# Autodesk Inventor assembly: project_maket
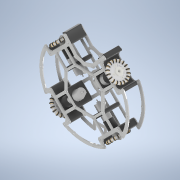
[picture p0: Inventor's stored thumbnail of the model, 180x180]
Saved by Autodesk Inventor 2020 (Build 240168000, 168)
## iProperties
Created: 2024-02-27
Part Number: project_maket
Document SubType Name: Assembly
Designer: 4s
Author: 4s
## Documents named in this file (9)
- C:\Users\4s\Documents\Inventor models\Asterisk\robot_v2\project_maket.iam
- C:\Users\4s\Documents\Inventor models\Asterisk\robot_v2\bottom_plate.ipt
- C:\Users\4s\Documents\Inventor models\Asterisk\robot_v2\motor mounts\mid_mount.ipt
- C:\Users\4s\Documents\Inventor models\Asterisk\robot_v2\motor mounts\left_motor_v2.ipt
- C:\Users\4s\Documents\Inventor models\Asterisk\robot_v2\motor mounts\right_motor_v2.ipt
- C:\Users\4s\Documents\Inventor models\Asterisk\robot_v2\motor mounts\back_motor_short.ipt
- C:\Users\4s\Documents\Inventor models\Asterisk\robot_v2\upper_plate.ipt
- C:\Users\4s\Documents\Inventor models\Asterisk\robot_v2\motor_body.ipt
- C:\Users\4s\Documents\Inventor models\Asterisk\robot_v2\GTF Robots 50mm Wheel.ipt
## Components (18 placed, 8 different names)
1. bottom_plate:1 — Совмещение:1, Совмещение:2, Заподлицо:1, Совмещение:3, Совмещение:4, Совмещение:5, Совмещение:6, Совмещение:7, Совмещение:8, Совмещение:9, Совмещение:10, Совмещение:11, Совмещение:12, Совмещение:13, Совмещение:14, Совмещение:15, Совмещение:16, Совмещение:17, Совмещение:18, Совмещение:19, Совмещение:20, Совмещение:21, Совмещение:22, Совмещение:23, Совмещение:24, Совмещение:25, Совмещение:26, Совмещение:27, Совмещение:28, Заподлицо:2
2. mid_mount:1 — Совмещение:3, Совмещение:4, Совмещение:5
3. mid_mount:2 — Совмещение:10, Совмещение:11, Совмещение:12
4. mid_mount:3 — Совмещение:8, Совмещение:9, Совмещение:13
5. mid_mount:4 — Совмещение:6, Совмещение:7, Совмещение:14
6. left_motor_v2:1 — Совмещение:21, Совмещение:22, Совмещение:23, Совмещение:31, Совмещение:32, Совмещение:38
7. right_motor_v2:1 — Совмещение:24, Совмещение:25, Совмещение:26, Совмещение:29, Совмещение:30, Совмещение:43, Совмещение:44
8. back_motor_short:1 — Совмещение:15, Совмещение:16, Совмещение:17, Совмещение:33, Совмещение:34, Совмещение:40
9. back_motor_short:2 — Совмещение:18, Совмещение:19, Совмещение:20, Совмещение:35, Совмещение:36, Совмещение:42
10. upper_plate:1 — Совмещение:27, Совмещение:28, Заподлицо:2
11. motor_body:1 — Совмещение:29, Совмещение:30
12. motor_body:2 — Совмещение:31, Совмещение:32, Совмещение:37
13. motor_body:3 — Совмещение:33, Совмещение:34, Совмещение:39
14. motor_body:4 — Совмещение:35, Совмещение:36, Совмещение:41
15. GTF Robots 50mm Wheel:1 — Совмещение:39, Совмещение:40
16. GTF Robots 50mm Wheel:2 — Совмещение:41, Совмещение:42
17. GTF Robots 50mm Wheel:3 — Совмещение:43, Совмещение:44
18. GTF Robots 50mm Wheel:4 — Совмещение:37, Совмещение:38
## Relationships (46: Mate 44, Flush 2)
- Совмещение:1 [Mate]: bottom_plate:1
- Совмещение:2 [Mate]: bottom_plate:1
- Заподлицо:1 [Flush]: bottom_plate:1
- Совмещение:3 [Mate]: bottom_plate:1 ↔ mid_mount:1
- Совмещение:4 [Mate]: bottom_plate:1 ↔ mid_mount:1
- Совмещение:5 [Mate]: bottom_plate:1 ↔ mid_mount:1
- Совмещение:6 [Mate]: bottom_plate:1 ↔ mid_mount:4
- Совмещение:7 [Mate]: bottom_plate:1 ↔ mid_mount:4
- Совмещение:8 [Mate]: bottom_plate:1 ↔ mid_mount:3
- Совмещение:9 [Mate]: bottom_plate:1 ↔ mid_mount:3
- Совмещение:10 [Mate]: bottom_plate:1 ↔ mid_mount:2
- Совмещение:11 [Mate]: bottom_plate:1 ↔ mid_mount:2
- Совмещение:12 [Mate]: bottom_plate:1 ↔ mid_mount:2
- Совмещение:13 [Mate]: bottom_plate:1 ↔ mid_mount:3
- Совмещение:14 [Mate]: bottom_plate:1 ↔ mid_mount:4
- Совмещение:15 [Mate]: bottom_plate:1 ↔ back_motor_short:1
- Совмещение:16 [Mate]: bottom_plate:1 ↔ back_motor_short:1
- Совмещение:17 [Mate]: bottom_plate:1 ↔ back_motor_short:1
- Совмещение:18 [Mate]: bottom_plate:1 ↔ back_motor_short:2
- Совмещение:19 [Mate]: bottom_plate:1 ↔ back_motor_short:2
- Совмещение:20 [Mate]: bottom_plate:1 ↔ back_motor_short:2
- Совмещение:21 [Mate]: bottom_plate:1 ↔ left_motor_v2:1
- Совмещение:22 [Mate]: bottom_plate:1 ↔ left_motor_v2:1
- Совмещение:23 [Mate]: bottom_plate:1 ↔ left_motor_v2:1
- Совмещение:24 [Mate]: bottom_plate:1 ↔ right_motor_v2:1
- Совмещение:25 [Mate]: bottom_plate:1 ↔ right_motor_v2:1
- Совмещение:26 [Mate]: bottom_plate:1 ↔ right_motor_v2:1
- Совмещение:27 [Mate] (35 mm): bottom_plate:1 ↔ upper_plate:1
- Совмещение:28 [Mate]: bottom_plate:1 ↔ upper_plate:1
- Заподлицо:2 [Flush]: bottom_plate:1 ↔ upper_plate:1
- Совмещение:29 [Mate]: right_motor_v2:1 ↔ motor_body:1
- Совмещение:30 [Mate]: right_motor_v2:1 ↔ motor_body:1
- Совмещение:31 [Mate]: left_motor_v2:1 ↔ motor_body:2
- Совмещение:32 [Mate]: left_motor_v2:1 ↔ motor_body:2
- Совмещение:33 [Mate]: back_motor_short:1 ↔ motor_body:3
- Совмещение:34 [Mate]: back_motor_short:1 ↔ motor_body:3
- Совмещение:35 [Mate]: back_motor_short:2 ↔ motor_body:4
- Совмещение:36 [Mate]: back_motor_short:2 ↔ motor_body:4
- Совмещение:37 [Mate]: motor_body:2 ↔ GTF Robots 50mm Wheel:4
- Совмещение:38 [Mate]: left_motor_v2:1 ↔ GTF Robots 50mm Wheel:4
- Совмещение:39 [Mate]: motor_body:3 ↔ GTF Robots 50mm Wheel:1
- Совмещение:40 [Mate]: back_motor_short:1 ↔ GTF Robots 50mm Wheel:1
- Совмещение:41 [Mate]: motor_body:4 ↔ GTF Robots 50mm Wheel:2
- Совмещение:42 [Mate]: back_motor_short:2 ↔ GTF Robots 50mm Wheel:2
- Совмещение:43 [Mate]: right_motor_v2:1 ↔ GTF Robots 50mm Wheel:3
- Совмещение:44 [Mate]: right_motor_v2:1 ↔ GTF Robots 50mm Wheel:3
